# Autodesk Inventor assembly: Router And Mount
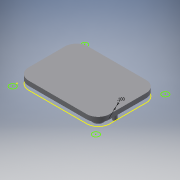
[picture p0: Inventor's stored thumbnail of the model, 180x180]
Saved by Autodesk Inventor 2016 (Build 200138000, 138)
## iProperties
Created: 2016-01-17
Part Number: Router And Mount
Document SubType Name: Assembly
Designer: Spooner
Author: Spooner
## Documents named in this file (3)
- C:\Users\Spooner\Documents\Inventor\2016 Radio Mount\Router And Mount.iam
- C:\Users\Spooner\Documents\Inventor\2016 Radio Mount\Router Bottom.ipt
- C:\Users\Spooner\Documents\Inventor\2016 Radio Mount\router mount.ipt
## Components (2 placed, 2 different names)
1. Router Bottom:1 — Flush:1
2. router mount:1 — Flush:1
## Relationships (1: Flush 1)
- Flush:1: Router Bottom:1 ↔ router mount:1
